# Autodesk Inventor assembly: Drive Assembly
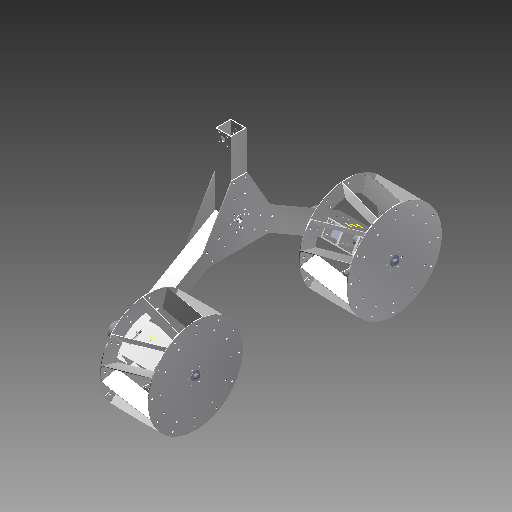
[picture p0: Inventor's stored thumbnail of the model, 512x512]
Saved by Autodesk Inventor 2019 (Build 230136000, 136)
## iProperties
Created: 2018-10-14
Part Number: Drive Assembly
Document SubType Name: Assembly
Designer: Adhik
Mass: 6827.49 g
Surface Area: 20406.1 cm^2
Volume: 2546.71 cm^3
Density: 2.68091 g/cm^3
Author: Adhik
## Documents named in this file (5)
- E:\CAD\Julie\Drive Assembly.iam
- E:\CAD\Julie\Outer Gusset Plate.ipt
- E:\CAD\Julie\Drive Arm.iam
- E:\CAD\Julie\Arm 8 inch.ipt
- E:\CAD\Julie\Arm Bearing.ipt
## Components (7 placed, 4 different names)
1. Outer Gusset Plate:1 — Flush:1, Flush:2, Mate:1, Mate:2, Mate:3, Mate:4, Mate:5, Mate:6, Mate:8, Mate:9, Mate:10, Insert:2
2. Outer Gusset Plate:2 — Flush:1, Flush:2, Mate:7, Insert:1
3. Drive Arm:1 [sub-assembly] — Mate:1, Mate:3, Mate:4, Mate:7
4. Drive Arm:2 [sub-assembly] — Mate:2, Mate:5, Mate:6
5. Arm 8 inch:1 — Mate:8, Mate:9, Mate:10
6. Arm Bearing:1 — Insert:2
7. Arm Bearing:2 — Insert:1
## Relationships (14: Mate 10, Flush 2, Insert 2)
- Flush:1: Outer Gusset Plate:1 ↔ Outer Gusset Plate:2
- Flush:2: Outer Gusset Plate:1 ↔ Outer Gusset Plate:2
- Mate:1: Outer Gusset Plate:1 ↔ Drive Arm:1
- Mate:2: Outer Gusset Plate:1 ↔ Drive Arm:2
- Mate:3: Outer Gusset Plate:1 ↔ Drive Arm:1
- Mate:4: Outer Gusset Plate:1 ↔ Drive Arm:1
- Mate:5: Outer Gusset Plate:1 ↔ Drive Arm:2
- Mate:6: Outer Gusset Plate:1 ↔ Drive Arm:2
- Mate:7: Outer Gusset Plate:2 ↔ Drive Arm:1
- Mate:8: Outer Gusset Plate:1 ↔ Arm 8 inch:1
- Mate:9: Outer Gusset Plate:1 ↔ Arm 8 inch:1
- Mate:10: Outer Gusset Plate:1 ↔ Arm 8 inch:1
- Insert:1: Outer Gusset Plate:2 ↔ Arm Bearing:2
- Insert:2: Outer Gusset Plate:1 ↔ Arm Bearing:1
